# Autodesk Inventor assembly: V2_Herramienta_Final
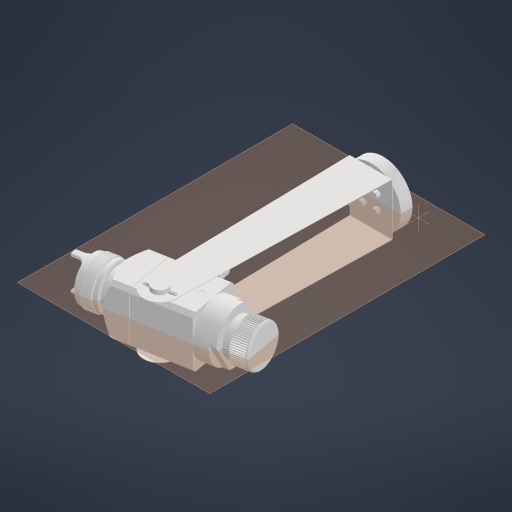
[picture p0: Inventor's stored thumbnail of the model, 512x512]
Saved by Autodesk Inventor 2024 (Build 280153000, 153)
## iProperties
Created: 2023-05-12
Part Number: V2_Herramienta_Final
Document SubType Name: Assembly
Designer: javie
Author: javie
## Documents named in this file (3)
- C:\Users\javie\Downloads\Herramienta\V2_Herramienta_Final.iam
- C:\Users\javie\Downloads\Herramienta\BaseH.ipt
- C:\Users\javie\Downloads\Herramienta\Herramienta_Final.iam
## Components (2 placed, 2 different names)
1. BaseH:1 — Insertar:1
2. Herramienta_Final:1 [sub-assembly] — Insertar:1
## Relationships (1: Insert 1)
- Insertar:1: BaseH:1 ↔ Herramienta_Final:1
